# Autodesk Inventor assembly: Frame0001
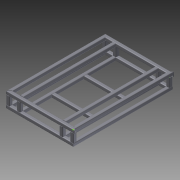
[picture p0: Inventor's stored thumbnail of the model, 180x180]
Saved by Autodesk Inventor 2013 (Build 170138000, 138)
## iProperties
Created: 2013-08-10
Part Number: Frame0001
Document SubType Name: Assembly
Designer: Creo
_FrameDoc: Frame Assembly
_Version: 15.0.0
Author: Creo
## Documents named in this file (46)
- E:\Robot Base Assembly\Frame\Frame0001.iam
- E:\Robot Base Assembly\Frame\Skeleton0001.ipt
- E:\Robot Base Assembly\Frame\ANSI 1-1_4x1-1_4x1_8 00000001.ipt
- ANSI 1-1_4x1-1_4x1_8 00000001.ipt
- E:\Robot Base Assembly\Frame\ANSI 1-1_4x1-1_4x1_8 00000002.ipt
- ANSI 1-1_4x1-1_4x1_8 00000002.ipt
- E:\Robot Base Assembly\Frame\ANSI 1-1_4x1-1_4x1_8 00000003.ipt
- ANSI 1-1_4x1-1_4x1_8 00000003.ipt
- E:\Robot Base Assembly\Frame\ANSI 1-1_4x1-1_4x1_8 00000004.ipt
- ANSI 1-1_4x1-1_4x1_8 00000004.ipt
- E:\Robot Base Assembly\Frame\ANSI 1-1_4x1-1_4x1_8 00000005.ipt
- ANSI 1-1_4x1-1_4x1_8 00000005.ipt
- E:\Robot Base Assembly\Frame\ANSI 1-1_4x1-1_4x1_8 00000006.ipt
- ANSI 1-1_4x1-1_4x1_8 00000006.ipt
- E:\Robot Base Assembly\Frame\ANSI 1-1_4x1-1_4x1_8 00000007.ipt
- ANSI 1-1_4x1-1_4x1_8 00000007.ipt
- E:\Robot Base Assembly\Frame\ANSI 1-1_4x1-1_4x1_8 00000008.ipt
- ANSI 1-1_4x1-1_4x1_8 00000008.ipt
- E:\Robot Base Assembly\Frame\ANSI 1-1_4x1-1_4x1_8 00000009.ipt
- ANSI 1-1_4x1-1_4x1_8 00000009.ipt
- E:\Robot Base Assembly\Frame\ANSI 1-1_4x1-1_4x1_8 00000010.ipt
- ANSI 1-1_4x1-1_4x1_8 00000010.ipt
- E:\Robot Base Assembly\Frame\ANSI 1-1_4x1-1_4x1_8 00000011.ipt
- ANSI 1-1_4x1-1_4x1_8 00000011.ipt
- E:\Robot Base Assembly\Frame\ANSI 1-1_4x1-1_4x1_8 00000012.ipt
- ANSI 1-1_4x1-1_4x1_8 00000012.ipt
- E:\Robot Base Assembly\Frame\ANSI 1-1_4x1-1_4x1_8 00000013.ipt
- ANSI 1-1_4x1-1_4x1_8 00000013.ipt
- E:\Robot Base Assembly\Frame\ANSI 1-1_4x1-1_4x1_8 00000014.ipt
- ANSI 1-1_4x1-1_4x1_8 00000014.ipt
- E:\Robot Base Assembly\Frame\ANSI 1-1_4x1-1_4x1_8 00000015.ipt
- ANSI 1-1_4x1-1_4x1_8 00000015.ipt
- E:\Robot Base Assembly\Frame\ANSI 1-1_4x1-1_4x1_8 00000016.ipt
- ANSI 1-1_4x1-1_4x1_8 00000016.ipt
- E:\Robot Base Assembly\Frame\ANSI 1-1_4x1-1_4x1_8 00000017.ipt
- ANSI 1-1_4x1-1_4x1_8 00000017.ipt
- E:\Robot Base Assembly\Frame\ANSI 1-1_4x1-1_4x1_8 00000018.ipt
- ANSI 1-1_4x1-1_4x1_8 00000018.ipt
- E:\Robot Base Assembly\Frame\ANSI 1-1_4x1-1_4x1_8 00000019.ipt
- ANSI 1-1_4x1-1_4x1_8 00000019.ipt
- E:\Robot Base Assembly\Frame\ANSI 1-1_4x1-1_4x1_8 00000020.ipt
- ANSI 1-1_4x1-1_4x1_8 00000020.ipt
- E:\Robot Base Assembly\Frame\ANSI 1-1_4x1-1_4x1_8 00000021.ipt
- ANSI 1-1_4x1-1_4x1_8 00000021.ipt
- E:\Robot Base Assembly\Frame\ANSI 1-1_4x1-1_4x1_8 00000022.ipt
- ANSI 1-1_4x1-1_4x1_8 00000022.ipt
## Components (23 placed, 23 different names)
1. Frame Reference Model
2. ANSI 1-1_4x1-1_4x1_8 00000001:1
3. ANSI 1-1_4x1-1_4x1_8 00000002:1 — Flush:1, Flush:2
4. ANSI 1-1_4x1-1_4x1_8 00000003:1
5. ANSI 1-1_4x1-1_4x1_8 00000004:1
6. ANSI 1-1_4x1-1_4x1_8 00000005:1
7. ANSI 1-1_4x1-1_4x1_8 00000006:1
8. ANSI 1-1_4x1-1_4x1_8 00000007:1
9. ANSI 1-1_4x1-1_4x1_8 00000008:1
10. ANSI 1-1_4x1-1_4x1_8 00000009:1 — Flush:1, Flush:2
11. ANSI 1-1_4x1-1_4x1_8 00000010:1
12. ANSI 1-1_4x1-1_4x1_8 00000011:1
13. ANSI 1-1_4x1-1_4x1_8 00000012:1
14. ANSI 1-1_4x1-1_4x1_8 00000013:1
15. ANSI 1-1_4x1-1_4x1_8 00000014:1
16. ANSI 1-1_4x1-1_4x1_8 00000015:1
17. ANSI 1-1_4x1-1_4x1_8 00000016:1
18. ANSI 1-1_4x1-1_4x1_8 00000017:1
19. ANSI 1-1_4x1-1_4x1_8 00000018:1
20. ANSI 1-1_4x1-1_4x1_8 00000019:1
21. ANSI 1-1_4x1-1_4x1_8 00000020:1
22. ANSI 1-1_4x1-1_4x1_8 00000021:1
23. ANSI 1-1_4x1-1_4x1_8 00000022:1
## Relationships (2: Flush 2)
- Flush:1: ANSI 1-1_4x1-1_4x1_8 00000002:1 ↔ ANSI 1-1_4x1-1_4x1_8 00000009:1
- Flush:2: ANSI 1-1_4x1-1_4x1_8 00000002:1 ↔ ANSI 1-1_4x1-1_4x1_8 00000009:1
